# Autodesk Inventor assembly: Rectangular Legs
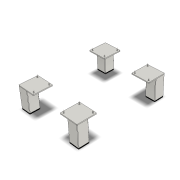
[picture p0: Inventor's stored thumbnail of the model, 180x180]
Saved by Autodesk Inventor 2024 (Build 280153000, 153)
## iProperties
RuleStatus: InUse
Created: 2023-03-08
Part Number: Rectangular Legs
Document SubType Name: Assembly
Designer: sauliusd
Author: sauliusd
## Documents named in this file (4)
- C:\W4INV 2024 Design\SMART HARDWARE\Legs\Rectangular Legs\Rectangular Legs.iam
- C:\W4INV 2024 Design\SMART HARDWARE\Legs\Rectangular Legs\Parts\Rectangular Legs Skeleton.ipt
- C:\W4INV 2022 Design\LIBRARY\Supports and legs\Legs\RECTANGULAR LEG.ipt
- C:\W4INV 2024 Design\_LIBRARY\Supports and legs\Legs\RECTANGULAR LEG\Rectangular leg H100.ipt
## Components (6 placed, 6 different names)
1. @Skeleton — Mate:1, Mate:2, Mate:3, Mate:4, Mate:5, Mate:6, Mate:7, Mate:8, Mate:10, Flush:1
2. Rectangular leg 1 — Mate:1, Mate:2
3. Rectangular leg 2 — Mate:3, Mate:4
4. Rectangular leg 3 — Mate:5, Mate:6
5. Rectangular leg 4 — Mate:7, Mate:8
6. Support Leg — Mate:9, Mate:10, Flush:1
## Relationships (11: Mate 10, Flush 1)
- Mate:1: @Skeleton ↔ Rectangular leg 1
- Mate:2: @Skeleton ↔ Rectangular leg 1
- Mate:3: @Skeleton ↔ Rectangular leg 2
- Mate:4: @Skeleton ↔ Rectangular leg 2
- Mate:5: @Skeleton ↔ Rectangular leg 3
- Mate:6: @Skeleton ↔ Rectangular leg 3
- Mate:7: @Skeleton ↔ Rectangular leg 4
- Mate:8: @Skeleton ↔ Rectangular leg 4
- Mate:9: Support Leg
- Mate:10 (-22.5 mm): @Skeleton ↔ Support Leg
- Flush:1 (22.5 mm): @Skeleton ↔ Support Leg
## Named parameters: Length = 400 mm, Depth = 300 mm, Shift_X = 0 mm, Shift_Y = 0 mm, Margins_X = 2 mm, Margins_Y = 2 mm, LegH = 100 mm
